# Autodesk Inventor assembly: Assembly1
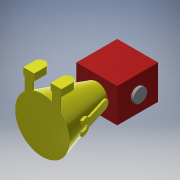
[picture p0: Inventor's stored thumbnail of the model, 180x180]
Saved by Autodesk Inventor 2019 (Build 230136000, 136)
## iProperties
Created: 2018-05-20
Part Number: Assembly1
Material: 一般
Document SubType Name: Assembly
Designer: uctom
Author: uctom
## Documents named in this file (4)
- C:\Users\uctom\OneDrive\デスクトップ\Assembly1.iam
- C:\Users\uctom\OneDrive\デスクトップ\body.ipt
- C:\Users\uctom\OneDrive\デスクトップ\head.ipt
- C:\Users\uctom\OneDrive\デスクトップ\ear.ipt
## Components (3 placed, 3 different names)
1. body:1 — フラッシュ:1
2. head:1 — フラッシュ:1, フラッシュ:2
3. ear:1 — フラッシュ:2
## Relationships (2: Flush 2)
- フラッシュ:1 [Flush]: body:1 ↔ head:1
- フラッシュ:2 [Flush]: head:1 ↔ ear:1
